# Autodesk Inventor assembly: SCARA
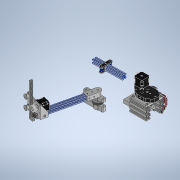
[picture p0: Inventor's stored thumbnail of the model, 180x180]
Saved by Autodesk Inventor 2022 (Build 260153000, 153)
## iProperties
Created: 2022-03-02
Part Number: SCARA
Document SubType Name: Assembly
Designer: JK
Author: JK
## Documents named in this file (7)
- C:\Users\JK\Documents\Inventor\ScaraNema\SCARA-3DP\Parts\SCARA.iam
- C:\Users\JK\Documents\Inventor\ScaraNema\SCARA-3DP\Parts\Shoulder\Shoulder base.iam
- C:\Users\JK\Documents\Inventor\ScaraNema\SCARA-3DP\Parts\Elbow\Elbow assembly.iam
- C:\Users\JK\Documents\Inventor\ScaraNema\SCARA-3DP\Parts\Z axis\Z assembly.iam
- C:\Users\JK\Documents\Inventor\ScaraNema\SCARA-3DP\Parts\Electronics\Electronics.iam
- C:\Users\JK\Documents\Inventor\ScaraNema\SCARA-3DP\Parts\Z axis\zupportenstop.ipt
- C:\Users\JK\Documents\Inventor\ScaraNema\SCARA-3DP\Parts\25T0397-001.ipt
## Components (6 placed, 6 different names)
1. Shoulder base:1 [sub-assembly] — Coincidencia:5, Coincidencia:6
2. Elbow assembly:1 [sub-assembly] — Coincidencia:5, Coincidencia:6, Coincidencia:7, Coincidencia:8, Coincidencia:9
3. Z assembly:1 [sub-assembly] — Coincidencia:7, Coincidencia:8, Coincidencia:9, Coincidencia:10, Nivelación:2, Nivelación:3
4. Electronics:1 [sub-assembly]
5. zupportenstop:1 — Coincidencia:10, Nivelación:2, Coincidencia:11, Coincidencia:12, Coincidencia:13
6. 25T0397-001:1 — Coincidencia:11, Coincidencia:12, Coincidencia:13, Nivelación:3
## Relationships (11: Mate 9, Flush 2)
- Coincidencia:5 [Mate]: Shoulder base:1 ↔ Elbow assembly:1
- Coincidencia:6 [Mate] (-30 mm): Shoulder base:1 ↔ Elbow assembly:1
- Coincidencia:7 [Mate]: Elbow assembly:1 ↔ Z assembly:1
- Coincidencia:8 [Mate] (0.15 mm): Elbow assembly:1 ↔ Z assembly:1
- Coincidencia:9 [Mate]: Elbow assembly:1 ↔ Z assembly:1
- Coincidencia:10 [Mate]: Z assembly:1 ↔ zupportenstop:1
- Nivelación:2 [Flush]: Z assembly:1 ↔ zupportenstop:1
- Coincidencia:11 [Mate]: zupportenstop:1 ↔ 25T0397-001:1
- Coincidencia:12 [Mate]: zupportenstop:1 ↔ 25T0397-001:1
- Coincidencia:13 [Mate]: zupportenstop:1 ↔ 25T0397-001:1
- Nivelación:3 [Flush] (5 mm): Z assembly:1 ↔ 25T0397-001:1
